# Autodesk Inventor assembly: rapoukBaseAssemblyv0
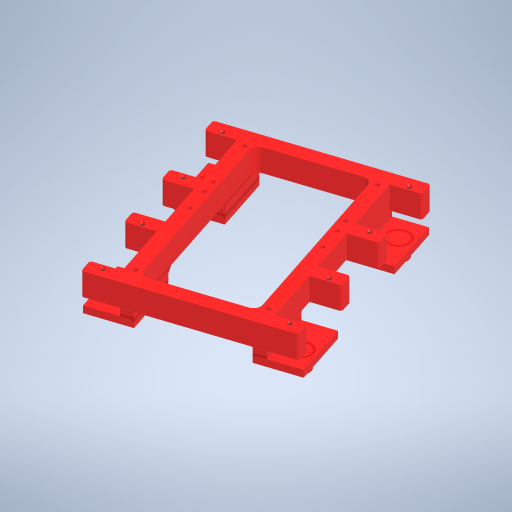
[picture p0: Inventor's stored thumbnail of the model, 512x512]
Saved by Autodesk Inventor 2024 (Build 280153000, 153)
## iProperties
Created: 2024-01-09
Part Number: rapoukBaseAssemblyv0
Document SubType Name: Weldment
Designer: Roman Suk
Weld Material: Welded Aluminum-6061
Author: Roman Suk
## Documents named in this file (5)
- C:\Users\Roman Suk\Documents\Ročníkovka SŠ\Technical documentation\Final1\rapoukBaseAssemblyv0.iam
- C:\Users\Roman Suk\Documents\Ročníkovka SŠ\Technical documentation\Final1\rapoukBasev5.ipt
- C:\Users\Roman Suk\Documents\Ročníkovka SŠ\Technical documentation\Final1\rapoukLegSupportv1.ipt
- C:\Users\Roman Suk\Documents\Ročníkovka SŠ\Technical documentation\Final1\rapoukLegBasev3.ipt
- C:\Users\Roman Suk\Documents\Ročníkovka SŠ\Technical documentation\Final1\rapoukLegPinv1.ipt
## Components (13 placed, 4 different names)
1. rapoukBasev5:1 — Mate:1, Mate:2, Mate:3, Mate:4, Mate:5, Mate:6, Mate:7, Mate:8, Flush:1, Flush:2, Flush:3, Flush:4
2. rapoukLegSupportv1:1 — Mate:4, Mate:8, Flush:4, Mate:11, Flush:9, Flush:10
3. rapoukLegSupportv1:2 — Mate:3, Mate:7, Flush:3, Mate:12, Flush:11, Flush:12
4. rapoukLegSupportv1:3 — Mate:2, Mate:6, Flush:2, Mate:9, Flush:5, Flush:6
5. rapoukLegSupportv1:4 — Mate:1, Mate:5, Flush:1, Mate:10, Flush:7, Flush:8
6. rapoukLegBasev3:1 — Mate:11, Flush:9, Flush:10, Flush:14, Tangent:1
7. rapoukLegBasev3:2 — Mate:12, Flush:11, Flush:12, Flush:15, Tangent:4
8. rapoukLegBasev3:3 — Mate:9, Flush:5, Flush:6, Flush:16, Tangent:3
9. rapoukLegBasev3:4 — Mate:10, Flush:7, Flush:8, Flush:13, Tangent:2
10. rapoukLegPinv1:1 — Flush:13, Tangent:2
11. rapoukLegPinv1:2 — Flush:14, Tangent:3
12. rapoukLegPinv1:3 — Flush:15, Tangent:4
13. rapoukLegPinv1:4 — Flush:16, Tangent:1
## Relationships (32: Flush 16, Mate 12, Tangent 4)
- Mate:1: rapoukBasev5:1 ↔ rapoukLegSupportv1:4
- Mate:2: rapoukBasev5:1 ↔ rapoukLegSupportv1:3
- Mate:3: rapoukBasev5:1 ↔ rapoukLegSupportv1:2
- Mate:4: rapoukBasev5:1 ↔ rapoukLegSupportv1:1
- Mate:5 (3.7 mm): rapoukBasev5:1 ↔ rapoukLegSupportv1:4
- Mate:6 (-3.7 mm): rapoukBasev5:1 ↔ rapoukLegSupportv1:3
- Mate:7 (-3.7 mm): rapoukBasev5:1 ↔ rapoukLegSupportv1:2
- Mate:8 (-3.7 mm): rapoukBasev5:1 ↔ rapoukLegSupportv1:1
- Flush:1: rapoukBasev5:1 ↔ rapoukLegSupportv1:4
- Flush:2: rapoukBasev5:1 ↔ rapoukLegSupportv1:3
- Flush:3: rapoukBasev5:1 ↔ rapoukLegSupportv1:2
- Flush:4: rapoukBasev5:1 ↔ rapoukLegSupportv1:1
- Mate:9: rapoukLegSupportv1:3 ↔ rapoukLegBasev3:3
- Flush:5: rapoukLegSupportv1:3 ↔ rapoukLegBasev3:3
- Flush:6: rapoukLegSupportv1:3 ↔ rapoukLegBasev3:3
- Mate:10: rapoukLegSupportv1:4 ↔ rapoukLegBasev3:4
- Flush:7: rapoukLegSupportv1:4 ↔ rapoukLegBasev3:4
- Flush:8: rapoukLegSupportv1:4 ↔ rapoukLegBasev3:4
- Mate:11: rapoukLegSupportv1:1 ↔ rapoukLegBasev3:1
- Flush:9: rapoukLegSupportv1:1 ↔ rapoukLegBasev3:1
- Flush:10: rapoukLegSupportv1:1 ↔ rapoukLegBasev3:1
- Mate:12: rapoukLegSupportv1:2 ↔ rapoukLegBasev3:2
- Flush:11: rapoukLegSupportv1:2 ↔ rapoukLegBasev3:2
- Flush:12: rapoukLegSupportv1:2 ↔ rapoukLegBasev3:2
- Flush:13: rapoukLegBasev3:4 ↔ rapoukLegPinv1:1
- Flush:14: rapoukLegBasev3:1 ↔ rapoukLegPinv1:2
- Flush:15: rapoukLegBasev3:2 ↔ rapoukLegPinv1:3
- Flush:16: rapoukLegBasev3:3 ↔ rapoukLegPinv1:4
- Tangent:1: rapoukLegBasev3:1 ↔ rapoukLegPinv1:4
- Tangent:2: rapoukLegBasev3:4 ↔ rapoukLegPinv1:1
- Tangent:3: rapoukLegBasev3:3 ↔ rapoukLegPinv1:2
- Tangent:4: rapoukLegBasev3:2 ↔ rapoukLegPinv1:3
